# Autodesk Inventor assembly: robot
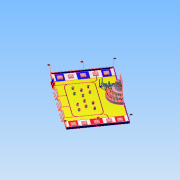
[picture p0: Inventor's stored thumbnail of the model, 180x180]
Saved by Autodesk Inventor 2013 (Build 170138000, 138)
## iProperties
Created: 2012-11-07
Part Number: robot
Document SubType Name: Assembly
Designer: Aegir
Author: Aegir
## Documents named in this file (13)
- C:\Users\Aegir\Documents\Robotik 2013\conception\robot.iam
- C:\Users\Aegir\Documents\Robotik 2013\conception\Base_Roulante_Ammovible.iam
- C:\Users\Aegir\Documents\Robotik 2013\conception\base robot.ipt
- C:\Users\Aegir\Documents\Robotik 2013\conception\profilé.ipt
- C:\Users\Aegir\Documents\Robotik 2013\conception\Composants importés\Raspberry_B1\Raspberry_B1.iam
- C:\Users\Aegir\Documents\Robotik 2013\conception\Composants importés\R220-MD22\R220-MD22.iam
- C:\Users\Aegir\Documents\Robotik 2013\conception\grosse batterie.ipt
- C:\Users\Aegir\Documents\Robotik 2013\conception\petite batterie.ipt
- C:\Users\Aegir\Documents\Robotik 2013\conception\verre.ipt
- C:\Users\Aegir\Documents\Robotik 2013\conception\tete_bras.ipt
- C:\Users\Aegir\Documents\Robotik 2013\conception\moteur euger 16_03.ipt
- C:\Users\Aegir\Documents\Robotik 2013\conception\tigemoteur.ipt
- C:\Users\Aegir\Documents\Robotik 2013\conception\Composants importés\table_2013\table_2013.iam
## Components (15 placed, 12 different names)
1. Base_Roulante_Ammovible:1 [sub-assembly] — Affleurement:1, Affleurement:2, Affleurement:5, Affleurement:8, Placage:17
2. base robot:1 — Affleurement:1, Affleurement:2, Affleurement:3, Affleurement:4, Placage:6, Tangente:6
3. profilé:1 — Affleurement:3, Affleurement:4, Affleurement:5, Placage:1, Angle:1, Placage:2, Placage:3, Angle:2, Angle:6
4. Raspberry_B1:1 [sub-assembly] — Placage:1, Angle:1
5. R220-MD22:1 [sub-assembly] — Placage:2, Placage:3
6. grosse batterie:1 — Placage:5, Affleurement:7, Placage:6, Tangente:2
7. grosse batterie:2 — Placage:4, Placage:5, Affleurement:6, Affleurement:7, Tangente:1, Tangente:2, Angle:2
8. petite batterie:1 — Placage:4, Affleurement:6, Tangente:1
9. verre:1 — Affleurement:8
10. tete_bras:1 — Placage:7, Angle:3, Placage:8, Angle:4, Placage:11, Placage:12, Placage:14, Placage:15, Angle:5, Placage:18, Tangente:7, Angle:6
11. moteur euger 16_03:1 — Placage:7, Angle:3, Affleurement:9, Placage:9, Placage:11, Placage:15, Tangente:5, Placage:16
12. moteur euger 16_03:2 — Placage:8, Angle:4, Placage:10, Placage:12, Tangente:4, Placage:13, Placage:14
13. tigemoteur:1 — Affleurement:9, Placage:9, Tangente:5, Placage:16
14. tigemoteur:2 — Placage:10, Tangente:4, Placage:13, Angle:5
15. table_2013:1 [sub-assembly] — Placage:17, Tangente:6, Placage:18, Tangente:7
## Relationships (39: Mate 18, Flush 9, Angle 6, Tangent 6)
- Affleurement:1 [Flush]: Base_Roulante_Ammovible:1 ↔ base robot:1
- Affleurement:2 [Flush]: Base_Roulante_Ammovible:1 ↔ base robot:1
- Affleurement:3 [Flush]: base robot:1 ↔ profilé:1
- Affleurement:4 [Flush]: base robot:1 ↔ profilé:1
- Affleurement:5 [Flush] (10 mm): Base_Roulante_Ammovible:1 ↔ profilé:1
- Placage:1 [Mate]: profilé:1 ↔ Raspberry_B1:1
- Angle:1 (180 deg): profilé:1 ↔ Raspberry_B1:1
- Placage:2 [Mate]: profilé:1 ↔ R220-MD22:1
- Placage:3 [Mate]: profilé:1 ↔ R220-MD22:1
- Placage:4 [Mate]: grosse batterie:2 ↔ petite batterie:1
- Placage:5 [Mate]: grosse batterie:1 ↔ grosse batterie:2
- Affleurement:6 [Flush]: grosse batterie:2 ↔ petite batterie:1
- Affleurement:7 [Flush]: grosse batterie:1 ↔ grosse batterie:2
- Placage:6 [Mate]: base robot:1 ↔ grosse batterie:1
- Tangente:1: grosse batterie:2 ↔ petite batterie:1
- Tangente:2: grosse batterie:1 ↔ grosse batterie:2
- Angle:2 (0 deg): profilé:1 ↔ grosse batterie:2
- Affleurement:8 [Flush]: Base_Roulante_Ammovible:1 ↔ verre:1
- Placage:7 [Mate]: tete_bras:1 ↔ moteur euger 16_03:1
- Angle:3 (25 deg): tete_bras:1 ↔ moteur euger 16_03:1
- Placage:8 [Mate]: tete_bras:1 ↔ moteur euger 16_03:2
- Affleurement:9 [Flush]: moteur euger 16_03:1 ↔ tigemoteur:1
- Placage:9 [Mate]: moteur euger 16_03:1 ↔ tigemoteur:1
- Angle:4 (25 deg): tete_bras:1 ↔ moteur euger 16_03:2
- Placage:10 [Mate]: moteur euger 16_03:2 ↔ tigemoteur:2
- Placage:11 [Mate]: tete_bras:1 ↔ moteur euger 16_03:1
- Placage:12 [Mate] (5 mm): tete_bras:1 ↔ moteur euger 16_03:2
- Tangente:4: moteur euger 16_03:2 ↔ tigemoteur:2
- Placage:13 [Mate]: moteur euger 16_03:2 ↔ tigemoteur:2
- Placage:14 [Mate]: tete_bras:1 ↔ moteur euger 16_03:2
- Placage:15 [Mate] (-10 mm): tete_bras:1 ↔ moteur euger 16_03:1
- Tangente:5: moteur euger 16_03:1 ↔ tigemoteur:1
- Placage:16 [Mate]: moteur euger 16_03:1 ↔ tigemoteur:1
- Angle:5 (60 deg): tete_bras:1 ↔ tigemoteur:2
- Placage:17 [Mate]: Base_Roulante_Ammovible:1 ↔ table_2013:1
- Tangente:6: base robot:1 ↔ table_2013:1
- Placage:18 [Mate] (20 mm): tete_bras:1 ↔ table_2013:1
- Tangente:7: tete_bras:1 ↔ table_2013:1
- Angle:6 (0 deg): profilé:1 ↔ tete_bras:1
